# Autodesk Inventor assembly: Inset hinge for aluminium frame
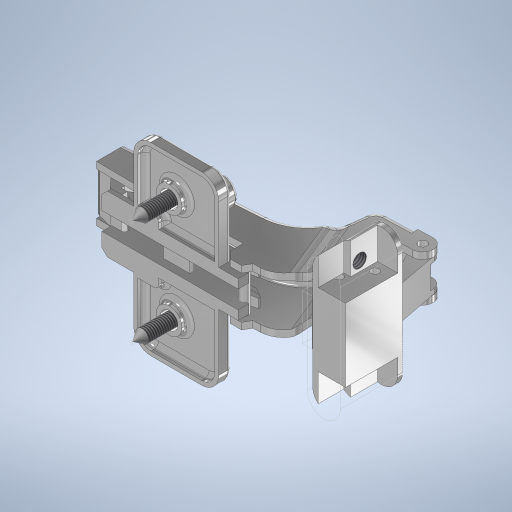
[picture p0: Inventor's stored thumbnail of the model, 512x512]
Saved by Autodesk Inventor 2024 (Build 280153000, 153)
## iProperties
Created: 2014-01-06
Part Number: Inset hinge for aluminium frame
Document SubType Name: Assembly
Designer: G. Kazokaitis
Author: G. Kazokaitis
## Documents named in this file (7)
- C:\W4INV 2024 Design\_LIBRARY\Hinges\HINGE FOR ALUMINIUM FRAME\Inset hinge for aluminium frame.iam
- C:\W4INV 2024 Design\LIBRARY\Hinges\Parts\Hinge for aluminium frame\Inset case.ipt
- C:\W4INV 2024 Design\LIBRARY\Hinges\Parts\Hinge for aluminium frame\Lever for inset hinge.ipt
- C:\W4INV 2024 Design\LIBRARY\Hinges\Parts\Hinge for aluminium frame\Linkage for inset hinge.ipt
- C:\W4INV 2024 Design\LIBRARY\Hinges\Parts\Hinge for aluminium frame\Mounting plate.ipt
- C:\W4INV 2024 Design\LIBRARY\Hinges\Parts\Hinge for aluminium frame\Cup.ipt
- C:\W4INV 2024 Design\LIBRARY\Hinges\HINGE FOR ALUMINIUM FRAME.iam
## Components (5 placed, 5 different names)
1. Mounting plate:1 — Flush:1, Flush:2, Mate:1, Flush:5, Mate:20, Mate:21
2. Cup:1 — Mate:26, Mate:27, Mate:28, Inset hinge opening angle
3. Inset case:1 — Flush:5, Mate:20, Mate:21, Mate:22, Mate:23, Mate:24, Mate:25, Inset hinge opening angle
4. Lever for inset hinge:1 — Mate:22, Mate:23, Mate:26, Mate:28
5. Linkage for inset hinge:1 — Mate:24, Mate:25, Mate:27
## Relationships (14: Mate 10, Flush 3, Angle 1)
- Flush:1: Mounting plate:1
- Flush:2: Mounting plate:1
- Mate:1: Mounting plate:1
- Flush:5: Mounting plate:1 ↔ Inset case:1
- Mate:20: Mounting plate:1 ↔ Inset case:1
- Mate:21: Mounting plate:1 ↔ Inset case:1
- Mate:22: Inset case:1 ↔ Lever for inset hinge:1
- Mate:23: Inset case:1 ↔ Lever for inset hinge:1
- Mate:24: Inset case:1 ↔ Linkage for inset hinge:1
- Mate:25: Inset case:1 ↔ Linkage for inset hinge:1
- Mate:26: Cup:1 ↔ Lever for inset hinge:1
- Mate:27: Cup:1 ↔ Linkage for inset hinge:1
- Mate:28 (1.9 mm): Cup:1 ↔ Lever for inset hinge:1
- Inset hinge opening angle [Angle] (180 deg): Cup:1 ↔ Inset case:1
## Named parameters: Offset_distance = 57 mm
